# Autodesk Inventor assembly: パネル型スカラアームMISUMIアルミフレーム作成Ver
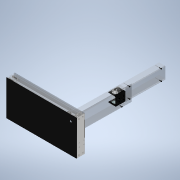
[picture p0: Inventor's stored thumbnail of the model, 180x180]
Saved by Autodesk Inventor 2022 (Build 260153000, 153)
## iProperties
Created: 2022-12-05
Part Number: パネル型スカラアームMISUMIアルミフレーム作成Ver
Document SubType Name: Assembly
Designer: tdn82
Author: tdn82
## Documents named in this file (29)
- C:\Users\tdn82\OneDrive\ドキュメント\Inventor\卒業研究パネル型スカラアーム\GrabCAD\panel-type-scalar-arm\パネル型スカラアーム\パネル型スカラアームMISUMIアルミフレーム作成Ver.iam
- C:\Users\tdn82\OneDrive\ドキュメント\Inventor\卒業研究パネル型スカラアーム\GrabCAD\panel-type-scalar-arm\パネル型スカラアーム\HFSF5-2040-180-LWH-RWH.ipt
- C:\Users\tdn82\OneDrive\ドキュメント\Inventor\卒業研究パネル型スカラアーム\GrabCAD\panel-type-scalar-arm\パネル型スカラアーム\HFSF5-2040-320-TPW.ipt
- C:\Users\tdn82\OneDrive\ドキュメント\Inventor\卒業研究パネル型スカラアーム\GrabCAD\panel-type-scalar-arm\パネル型スカラアーム\後ろカバー.ipt
- C:\Users\tdn82\OneDrive\ドキュメント\Inventor\卒業研究パネル型スカラアーム\GrabCAD\panel-type-scalar-arm\パネル型スカラアーム\サーボモータ固定用１軸目.ipt
- C:\Users\tdn82\OneDrive\ドキュメント\Inventor\卒業研究パネル型スカラアーム\GrabCAD\panel-type-scalar-arm\パネル型スカラアーム\サーボモータB3M-SC-1170-AB3M1100_scale.ipt
- C:\Users\tdn82\OneDrive\ドキュメント\Inventor\卒業研究パネル型スカラアーム\GrabCAD\panel-type-scalar-arm\パネル型スカラアーム\サーボ固定パーツ３Dプリンタ出力実験\サーボモータ固定用２軸目3mm改.ipt
- C:\Users\tdn82\OneDrive\ドキュメント\Inventor\卒業研究パネル型スカラアーム\GrabCAD\panel-type-scalar-arm\パネル型スカラアーム\横長2ndフラットバー上 アルミフレーム用.ipt
- C:\Users\tdn82\OneDrive\ドキュメント\Inventor\卒業研究パネル型スカラアーム\GrabCAD\panel-type-scalar-arm\パネル型スカラアーム\前カバー中盤左アーム固定.ipt
- C:\Users\tdn82\OneDrive\ドキュメント\Inventor\卒業研究パネル型スカラアーム\GrabCAD\panel-type-scalar-arm\パネル型スカラアーム\アルミフリーホーン02137_AluminumFreeHornWithBearing_B3M_6000.ipt
- C:\Users\tdn82\OneDrive\ドキュメント\Inventor\卒業研究パネル型スカラアーム\GrabCAD\panel-type-scalar-arm\パネル型スカラアーム\横長3rdフラットバー下.ipt
- C:\Users\tdn82\OneDrive\ドキュメント\Inventor\卒業研究パネル型スカラアーム\GrabCAD\panel-type-scalar-arm\パネル型スカラアーム\横長2ndフラットバー下 アルミフレーム用.ipt
- C:\Users\tdn82\OneDrive\ドキュメント\Inventor\卒業研究パネル型スカラアーム\GrabCAD\panel-type-scalar-arm\パネル型スカラアーム\前カバー中段右.ipt
- C:\Users\tdn82\OneDrive\ドキュメント\Inventor\卒業研究パネル型スカラアーム\GrabCAD\panel-type-scalar-arm\パネル型スカラアーム\前上カバーサーボ隠し.ipt
- C:\Users\tdn82\OneDrive\ドキュメント\Inventor\卒業研究パネル型スカラアーム\GrabCAD\panel-type-scalar-arm\パネル型スカラアーム\前下カバーサーボ隠し.ipt
- C:\Users\tdn82\OneDrive\ドキュメント\Inventor\卒業研究パネル型スカラアーム\GrabCAD\panel-type-scalar-arm\パネル型スカラアーム\ベアリング.ipt
- C:\Users\tdn82\OneDrive\ドキュメント\Inventor\卒業研究パネル型スカラアーム\GrabCAD\panel-type-scalar-arm\パネル型スカラアーム\シャフト.ipt
- C:\Users\tdn82\OneDrive\ドキュメント\Inventor\卒業研究パネル型スカラアーム\GrabCAD\panel-type-scalar-arm\パネル型スカラアーム\シャフトカラー.ipt
- C:\Users\tdn82\OneDrive\ドキュメント\Inventor\卒業研究パネル型スカラアーム\GrabCAD\panel-type-scalar-arm\パネル型スカラアーム\三段目アクリル板.ipt
- C:\Users\tdn82\OneDrive\ドキュメント\Inventor\卒業研究パネル型スカラアーム\GrabCAD\panel-type-scalar-arm\パネル型スカラアーム\シャフトカラー.iam
- C:\Users\tdn82\OneDrive\ドキュメント\Inventor\卒業研究パネル型スカラアーム\GrabCAD\panel-type-scalar-arm\パネル型スカラアーム\HFSF5-2040-180-LWH-RWH Left.ipt
- C:\Users\tdn82\OneDrive\ドキュメント\Inventor\卒業研究パネル型スカラアーム\GrabCAD\panel-type-scalar-arm\パネル型スカラアーム\HFS5-2040-180-Z5-YA10-YB170-Left.ipt
- C:\Users\tdn82\OneDrive\ドキュメント\Inventor\卒業研究パネル型スカラアーム\GrabCAD\panel-type-scalar-arm\パネル型スカラアーム\CBE5-20.ipt
- C:\Users\tdn82\OneDrive\ドキュメント\Inventor\卒業研究パネル型スカラアーム\GrabCAD\panel-type-scalar-arm\パネル型スカラアーム\CSPPN-ST-M3-6_STEP_AP203AP214\CSPPN-STC-M3-6CSPPN-ST-M3-6_203.ipt
- C:\Users\tdn82\OneDrive\ドキュメント\Inventor\卒業研究パネル型スカラアーム\GrabCAD\panel-type-scalar-arm\パネル型スカラアーム\CBE3-20.ipt
- C:\Users\tdn82\OneDrive\ドキュメント\Inventor\卒業研究パネル型スカラアーム\GrabCAD\panel-type-scalar-arm\パネル型スカラアーム\CSPSL-ST3W-M2_6-10_STEP_AP203AP214\サーボホーンとアーム固定するねじCSPSL-ST3W-M2_6-10_203.ipt
- C:\Users\tdn82\OneDrive\ドキュメント\Inventor\卒業研究パネル型スカラアーム\GrabCAD\panel-type-scalar-arm\パネル型スカラアーム\CSPPN-ST-M2_6-18_STEP_AP203AP214\CSPPN-ST-M2_6-18_203.ipt
- C:\Users\tdn82\OneDrive\ドキュメント\Inventor\卒業研究パネル型スカラアーム\GrabCAD\panel-type-scalar-arm\パネル型スカラアーム\CSPPN-ST-M3-6_STEP_AP203AP214\CSPPN-STC-M3-6CSPPN-ST-M3-10_203 - コピー.ipt
- C:\Users\tdn82\OneDrive\ドキュメント\Inventor\卒業研究パネル型スカラアーム\GrabCAD\panel-type-scalar-arm\パネル型スカラアーム\HFSF5-2040-180-LMH-RMH.ipt
## Components (69 placed, 27 different names)
1. HFSF5-2040-180-LWH-RWH:2 — 挿入:5, 挿入:7, メイト:4, フラッシュ:1, メイト:12, メイト:14, メイト:26, フラッシュ:4, 挿入:39, 挿入:40
2. HFSF5-2040-320-TPW:1 — 挿入:5, 挿入:7, メイト:1, メイト:5, メイト:13, 挿入:38, 挿入:44, 挿入:92
3. HFSF5-2040-320-TPW:2 — 挿入:39, 挿入:40, 挿入:41, 挿入:45, 挿入:46, 挿入:93
4. 後ろカバー:1 — メイト:1, メイト:26, フラッシュ:4
5. サーボモータ固定用１軸目:1 — 挿入:11, 挿入:12, 挿入:13, メイト:4, フラッシュ:1, 挿入:78, 挿入:79, 挿入:80
6. サーボモータB3M-SC-1170-AB3M1100_scale:1 — 挿入:11, 挿入:12, 挿入:13, メイト:5, 挿入:14
7. サーボモータ固定用２軸目3mm改:1 — 挿入:15, 挿入:16, 挿入:18, 挿入:19, 挿入:75, 挿入:76, 挿入:77
8. 横長2ndフラットバー上 アルミフレーム用:1 — 挿入:14, メイト:7, フラッシュ:3, メイト:19, 挿入:67, 挿入:68, 挿入:69, 挿入:70
9. 前カバー中盤左アーム固定:1 — メイト:7, 挿入:15, 挿入:16, 挿入:23, 挿入:24, フラッシュ:3, メイト:19, 挿入:72, 挿入:73, 挿入:74, 挿入:81, 挿入:82, 挿入:83, 挿入:84, 挿入:91, 角度:1
10. サーボモータB3M-SC-1170-AB3M1100_scale:2 — 挿入:17, 挿入:18, 挿入:19, メイト:22, 挿入:32
11. アルミフリーホーン02137_AluminumFreeHornWithBearing_B3M_6000:1 — 挿入:17, 挿入:30, 挿入:31
12. 横長3rdフラットバー下:1 — フラッシュ:2, メイト:22, 挿入:32, メイト:25, 挿入:59, 挿入:60, 挿入:61, 挿入:62
13. 横長3rdフラットバー下:2 — フラッシュ:2, 挿入:30, 挿入:31, メイト:23, メイト:24, 挿入:63, 挿入:64, 挿入:65, 挿入:66
14. 横長2ndフラットバー下 アルミフレーム用:1 — 挿入:23, 挿入:24, 挿入:26
15. 前カバー中段右:1 — メイト:12, メイト:15, メイト:16, メイト:17, メイト:18
16. 前上カバーサーボ隠し:1 — メイト:13, メイト:14, メイト:15, メイト:16
17. 前下カバーサーボ隠し:1 — メイト:17, メイト:18
18. ベアリング:1 — 挿入:26, 挿入:35
19. シャフト:1 — 挿入:36
20. シャフトカラー:2 — 挿入:35, 挿入:36, 挿入:37
21. 三段目アクリル板:1 — メイト:23, メイト:24, メイト:25, 挿入:85, 挿入:86, 挿入:87, 挿入:88, 角度:1
22. シャフトカラー:3 [sub-assembly] — 挿入:37, 挿入:46, 挿入:89, 挿入:90
23. HFSF5-2040-180-LWH-RWH Left:1 — 挿入:38, 挿入:41
24. HFS5-2040-180-Z5-YA10-YB170-Left:1 — 挿入:44, 挿入:45, 挿入:47, 挿入:48, 挿入:49, 挿入:50
25. CBE5-20:1 — 挿入:48
26. CBE5-20:2 — 挿入:47
27. CBE5-20:3 — 挿入:49
28. CBE5-20:4 — 挿入:50
29. CBE5-20:5 — 挿入:95
30. CBE5-20:6 — 挿入:94
31. CBE5-20:7 — 挿入:98
32. CBE5-20:8 — 挿入:97
33. CBE3-20:1 — 挿入:101
34. CBE3-20:2 — 挿入:102
35. CBE3-20:3 — 挿入:99
36. CBE3-20:4 — 挿入:100
37. サーボホーンとアーム固定するねじCSPSL-ST3W-M2_6-10_203:1 — 挿入:59
38. サーボホーンとアーム固定するねじCSPSL-ST3W-M2_6-10_203:2 — 挿入:61
39. サーボホーンとアーム固定するねじCSPSL-ST3W-M2_6-10_203:3 — 挿入:62
40. サーボホーンとアーム固定するねじCSPSL-ST3W-M2_6-10_203:4 — 挿入:60
41. サーボホーンとアーム固定するねじCSPSL-ST3W-M2_6-10_203:5 — 挿入:68
42. サーボホーンとアーム固定するねじCSPSL-ST3W-M2_6-10_203:6 — 挿入:67
43. サーボホーンとアーム固定するねじCSPSL-ST3W-M2_6-10_203:7 — 挿入:69
44. サーボホーンとアーム固定するねじCSPSL-ST3W-M2_6-10_203:8 — 挿入:70
45. サーボホーンとアーム固定するねじCSPSL-ST3W-M2_6-10_203:9 — 挿入:63
46. サーボホーンとアーム固定するねじCSPSL-ST3W-M2_6-10_203:10 — 挿入:64
47. サーボホーンとアーム固定するねじCSPSL-ST3W-M2_6-10_203:11 — 挿入:66
48. サーボホーンとアーム固定するねじCSPSL-ST3W-M2_6-10_203:12 — 挿入:65
49. CSPPN-STC-M3-6CSPPN-ST-M3-6_203:2 — 挿入:72
50. CSPPN-STC-M3-6CSPPN-ST-M3-6_203:3 — 挿入:74
51. CSPPN-STC-M3-6CSPPN-ST-M3-6_203:4 — 挿入:73
52. CSPPN-ST-M2_6-18_203:2 — 挿入:77
53. CSPPN-ST-M2_6-18_203:3 — 挿入:76
54. CSPPN-ST-M2_6-18_203:4 — 挿入:75
55. CSPPN-ST-M2_6-18_203:5 — 挿入:78
56. CSPPN-ST-M2_6-18_203:6 — 挿入:80
57. CSPPN-ST-M2_6-18_203:8 — 挿入:79
58. CSPPN-STC-M3-6CSPPN-ST-M3-10_203 - コピー:1 — 挿入:81
59. CSPPN-STC-M3-6CSPPN-ST-M3-10_203 - コピー:2 — 挿入:82
60. CSPPN-STC-M3-6CSPPN-ST-M3-10_203 - コピー:3 — 挿入:89
61. CSPPN-STC-M3-6CSPPN-ST-M3-10_203 - コピー:4 — 挿入:85
62. CSPPN-STC-M3-6CSPPN-ST-M3-10_203 - コピー:5 — 挿入:83
63. CSPPN-STC-M3-6CSPPN-ST-M3-10_203 - コピー:6 — 挿入:84
64. CSPPN-STC-M3-6CSPPN-ST-M3-10_203 - コピー:7 — 挿入:86
65. CSPPN-STC-M3-6CSPPN-ST-M3-10_203 - コピー:8 — 挿入:87
66. CSPPN-STC-M3-6CSPPN-ST-M3-10_203 - コピー:9 — 挿入:90
67. CSPPN-STC-M3-6CSPPN-ST-M3-10_203 - コピー:10 — 挿入:88
68. CSPPN-STC-M3-6CSPPN-ST-M3-6_203:5 — 挿入:91
69. HFSF5-2040-180-LMH-RMH:1 — 挿入:92, 挿入:93, 挿入:94, 挿入:95, 挿入:97, 挿入:98, 挿入:99, 挿入:100, 挿入:101, 挿入:102
## Relationships (95: Insert 73, Mate 17, Flush 4, Angle 1)
- 挿入:5 [Insert]: HFSF5-2040-180-LWH-RWH:2 ↔ HFSF5-2040-320-TPW:1
- 挿入:7 [Insert]: HFSF5-2040-180-LWH-RWH:2 ↔ HFSF5-2040-320-TPW:1
- メイト:1 [Mate]: HFSF5-2040-320-TPW:1 ↔ 後ろカバー:1
- 挿入:11 [Insert]: サーボモータ固定用１軸目:1 ↔ サーボモータB3M-SC-1170-AB3M1100_scale:1
- 挿入:12 [Insert]: サーボモータ固定用１軸目:1 ↔ サーボモータB3M-SC-1170-AB3M1100_scale:1
- 挿入:13 [Insert]: サーボモータ固定用１軸目:1 ↔ サーボモータB3M-SC-1170-AB3M1100_scale:1
- メイト:4 [Mate]: HFSF5-2040-180-LWH-RWH:2 ↔ サーボモータ固定用１軸目:1
- フラッシュ:1 [Flush]: HFSF5-2040-180-LWH-RWH:2 ↔ サーボモータ固定用１軸目:1
- メイト:5 [Mate] (0.5 mm): HFSF5-2040-320-TPW:1 ↔ サーボモータB3M-SC-1170-AB3M1100_scale:1
- 挿入:14 [Insert]: サーボモータB3M-SC-1170-AB3M1100_scale:1 ↔ 横長2ndフラットバー上 アルミフレーム用:1
- メイト:7 [Mate]: 横長2ndフラットバー上 アルミフレーム用:1 ↔ 前カバー中盤左アーム固定:1
- 挿入:15 [Insert]: サーボモータ固定用２軸目3mm改:1 ↔ 前カバー中盤左アーム固定:1
- 挿入:16 [Insert]: サーボモータ固定用２軸目3mm改:1 ↔ 前カバー中盤左アーム固定:1
- 挿入:17 [Insert]: サーボモータB3M-SC-1170-AB3M1100_scale:2 ↔ アルミフリーホーン02137_AluminumFreeHornWithBearing_B3M_6000:1
- 挿入:18 [Insert]: サーボモータ固定用２軸目3mm改:1 ↔ サーボモータB3M-SC-1170-AB3M1100_scale:2
- 挿入:19 [Insert]: サーボモータ固定用２軸目3mm改:1 ↔ サーボモータB3M-SC-1170-AB3M1100_scale:2
- フラッシュ:2 [Flush]: 横長3rdフラットバー下:1 ↔ 横長3rdフラットバー下:2
- 挿入:23 [Insert]: 前カバー中盤左アーム固定:1 ↔ 横長2ndフラットバー下 アルミフレーム用:1
- 挿入:24 [Insert]: 前カバー中盤左アーム固定:1 ↔ 横長2ndフラットバー下 アルミフレーム用:1
- メイト:12 [Mate]: HFSF5-2040-180-LWH-RWH:2 ↔ 前カバー中段右:1
- メイト:13 [Mate] (-1 mm): HFSF5-2040-320-TPW:1 ↔ 前上カバーサーボ隠し:1
- メイト:14 [Mate] (-1 mm): HFSF5-2040-180-LWH-RWH:2 ↔ 前上カバーサーボ隠し:1
- メイト:15 [Mate]: 前カバー中段右:1 ↔ 前上カバーサーボ隠し:1
- メイト:16 [Mate]: 前カバー中段右:1 ↔ 前上カバーサーボ隠し:1
- メイト:17 [Mate]: 前カバー中段右:1 ↔ 前下カバーサーボ隠し:1
- メイト:18 [Mate]: 前カバー中段右:1 ↔ 前下カバーサーボ隠し:1
- フラッシュ:3 [Flush] (29 mm): 横長2ndフラットバー上 アルミフレーム用:1 ↔ 前カバー中盤左アーム固定:1
- メイト:19 [Mate]: 横長2ndフラットバー上 アルミフレーム用:1 ↔ 前カバー中盤左アーム固定:1
- 挿入:26 [Insert]: 横長2ndフラットバー下 アルミフレーム用:1 ↔ ベアリング:1
- メイト:22 [Mate]: サーボモータB3M-SC-1170-AB3M1100_scale:2 ↔ 横長3rdフラットバー下:1
- 挿入:30 [Insert]: アルミフリーホーン02137_AluminumFreeHornWithBearing_B3M_6000:1 ↔ 横長3rdフラットバー下:2
- 挿入:31 [Insert]: アルミフリーホーン02137_AluminumFreeHornWithBearing_B3M_6000:1 ↔ 横長3rdフラットバー下:2
- 挿入:32 [Insert]: サーボモータB3M-SC-1170-AB3M1100_scale:2 ↔ 横長3rdフラットバー下:1
- メイト:23 [Mate]: 横長3rdフラットバー下:2 ↔ 三段目アクリル板:1
- メイト:24 [Mate]: 横長3rdフラットバー下:2 ↔ 三段目アクリル板:1
- メイト:25 [Mate]: 横長3rdフラットバー下:1 ↔ 三段目アクリル板:1
- メイト:26 [Mate]: HFSF5-2040-180-LWH-RWH:2 ↔ 後ろカバー:1
- フラッシュ:4 [Flush]: HFSF5-2040-180-LWH-RWH:2 ↔ 後ろカバー:1
- 挿入:35 [Insert]: ベアリング:1 ↔ シャフトカラー:2
- 挿入:36 [Insert] (-5 mm): シャフト:1 ↔ シャフトカラー:2
- 挿入:37 [Insert] (2 mm): シャフトカラー:2 ↔ シャフトカラー:3
- 挿入:38 [Insert]: HFSF5-2040-320-TPW:1 ↔ HFSF5-2040-180-LWH-RWH Left:1
- 挿入:39 [Insert]: HFSF5-2040-180-LWH-RWH:2 ↔ HFSF5-2040-320-TPW:2
- 挿入:40 [Insert]: HFSF5-2040-180-LWH-RWH:2 ↔ HFSF5-2040-320-TPW:2
- 挿入:41 [Insert]: HFSF5-2040-320-TPW:2 ↔ HFSF5-2040-180-LWH-RWH Left:1
- 挿入:44 [Insert] (6 mm): HFSF5-2040-320-TPW:1 ↔ HFS5-2040-180-Z5-YA10-YB170-Left:1
- 挿入:45 [Insert] (6 mm): HFSF5-2040-320-TPW:2 ↔ HFS5-2040-180-Z5-YA10-YB170-Left:1
- 挿入:46 [Insert]: HFSF5-2040-320-TPW:2 ↔ シャフトカラー:3
- 挿入:47 [Insert]: HFS5-2040-180-Z5-YA10-YB170-Left:1 ↔ CBE5-20:2
- 挿入:48 [Insert]: HFS5-2040-180-Z5-YA10-YB170-Left:1 ↔ CBE5-20:1
- 挿入:49 [Insert]: HFS5-2040-180-Z5-YA10-YB170-Left:1 ↔ CBE5-20:3
- 挿入:50 [Insert]: HFS5-2040-180-Z5-YA10-YB170-Left:1 ↔ CBE5-20:4
- 挿入:59 [Insert]: 横長3rdフラットバー下:1 ↔ サーボホーンとアーム固定するねじCSPSL-ST3W-M2_6-10_203:1
- 挿入:60 [Insert]: 横長3rdフラットバー下:1 ↔ サーボホーンとアーム固定するねじCSPSL-ST3W-M2_6-10_203:4
- 挿入:61 [Insert]: 横長3rdフラットバー下:1 ↔ サーボホーンとアーム固定するねじCSPSL-ST3W-M2_6-10_203:2
- 挿入:62 [Insert]: 横長3rdフラットバー下:1 ↔ サーボホーンとアーム固定するねじCSPSL-ST3W-M2_6-10_203:3
- 挿入:63 [Insert]: 横長3rdフラットバー下:2 ↔ サーボホーンとアーム固定するねじCSPSL-ST3W-M2_6-10_203:9
- 挿入:64 [Insert]: 横長3rdフラットバー下:2 ↔ サーボホーンとアーム固定するねじCSPSL-ST3W-M2_6-10_203:10
- 挿入:65 [Insert]: 横長3rdフラットバー下:2 ↔ サーボホーンとアーム固定するねじCSPSL-ST3W-M2_6-10_203:12
- 挿入:66 [Insert]: 横長3rdフラットバー下:2 ↔ サーボホーンとアーム固定するねじCSPSL-ST3W-M2_6-10_203:11
- 挿入:67 [Insert]: 横長2ndフラットバー上 アルミフレーム用:1 ↔ サーボホーンとアーム固定するねじCSPSL-ST3W-M2_6-10_203:6
- 挿入:68 [Insert]: 横長2ndフラットバー上 アルミフレーム用:1 ↔ サーボホーンとアーム固定するねじCSPSL-ST3W-M2_6-10_203:5
- 挿入:69 [Insert]: 横長2ndフラットバー上 アルミフレーム用:1 ↔ サーボホーンとアーム固定するねじCSPSL-ST3W-M2_6-10_203:7
- 挿入:70 [Insert]: 横長2ndフラットバー上 アルミフレーム用:1 ↔ サーボホーンとアーム固定するねじCSPSL-ST3W-M2_6-10_203:8
- 挿入:72 [Insert]: 前カバー中盤左アーム固定:1 ↔ CSPPN-STC-M3-6CSPPN-ST-M3-6_203:2
- 挿入:73 [Insert]: 前カバー中盤左アーム固定:1 ↔ CSPPN-STC-M3-6CSPPN-ST-M3-6_203:4
- 挿入:74 [Insert]: 前カバー中盤左アーム固定:1 ↔ CSPPN-STC-M3-6CSPPN-ST-M3-6_203:3
- 挿入:75 [Insert]: サーボモータ固定用２軸目3mm改:1 ↔ CSPPN-ST-M2_6-18_203:4
- 挿入:76 [Insert]: サーボモータ固定用２軸目3mm改:1 ↔ CSPPN-ST-M2_6-18_203:3
- 挿入:77 [Insert]: サーボモータ固定用２軸目3mm改:1 ↔ CSPPN-ST-M2_6-18_203:2
- 挿入:78 [Insert]: サーボモータ固定用１軸目:1 ↔ CSPPN-ST-M2_6-18_203:5
- 挿入:79 [Insert]: サーボモータ固定用１軸目:1 ↔ CSPPN-ST-M2_6-18_203:8
- 挿入:80 [Insert]: サーボモータ固定用１軸目:1 ↔ CSPPN-ST-M2_6-18_203:6
- 挿入:81 [Insert]: 前カバー中盤左アーム固定:1 ↔ CSPPN-STC-M3-6CSPPN-ST-M3-10_203 - コピー:1
- 挿入:82 [Insert]: 前カバー中盤左アーム固定:1 ↔ CSPPN-STC-M3-6CSPPN-ST-M3-10_203 - コピー:2
- 挿入:83 [Insert]: 前カバー中盤左アーム固定:1 ↔ CSPPN-STC-M3-6CSPPN-ST-M3-10_203 - コピー:5
- 挿入:84 [Insert]: 前カバー中盤左アーム固定:1 ↔ CSPPN-STC-M3-6CSPPN-ST-M3-10_203 - コピー:6
- 挿入:85 [Insert]: 三段目アクリル板:1 ↔ CSPPN-STC-M3-6CSPPN-ST-M3-10_203 - コピー:4
- 挿入:86 [Insert]: 三段目アクリル板:1 ↔ CSPPN-STC-M3-6CSPPN-ST-M3-10_203 - コピー:7
- 挿入:87 [Insert]: 三段目アクリル板:1 ↔ CSPPN-STC-M3-6CSPPN-ST-M3-10_203 - コピー:8
- 挿入:88 [Insert]: 三段目アクリル板:1 ↔ CSPPN-STC-M3-6CSPPN-ST-M3-10_203 - コピー:10
- 挿入:89 [Insert]: シャフトカラー:3 ↔ CSPPN-STC-M3-6CSPPN-ST-M3-10_203 - コピー:3
- 挿入:90 [Insert]: シャフトカラー:3 ↔ CSPPN-STC-M3-6CSPPN-ST-M3-10_203 - コピー:9
- 挿入:91 [Insert]: 前カバー中盤左アーム固定:1 ↔ CSPPN-STC-M3-6CSPPN-ST-M3-6_203:5
- 角度:1 [Angle] (0 deg): 前カバー中盤左アーム固定:1 ↔ 三段目アクリル板:1
- 挿入:92 [Insert]: HFSF5-2040-320-TPW:1 ↔ HFSF5-2040-180-LMH-RMH:1
- 挿入:93 [Insert]: HFSF5-2040-320-TPW:2 ↔ HFSF5-2040-180-LMH-RMH:1
- 挿入:94 [Insert]: CBE5-20:6 ↔ HFSF5-2040-180-LMH-RMH:1
- 挿入:95 [Insert]: CBE5-20:5 ↔ HFSF5-2040-180-LMH-RMH:1
- 挿入:97 [Insert]: CBE5-20:8 ↔ HFSF5-2040-180-LMH-RMH:1
- 挿入:98 [Insert]: CBE5-20:7 ↔ HFSF5-2040-180-LMH-RMH:1
- 挿入:99 [Insert]: CBE3-20:3 ↔ HFSF5-2040-180-LMH-RMH:1
- 挿入:100 [Insert]: CBE3-20:4 ↔ HFSF5-2040-180-LMH-RMH:1
- 挿入:101 [Insert]: CBE3-20:1 ↔ HFSF5-2040-180-LMH-RMH:1
- 挿入:102 [Insert]: CBE3-20:2 ↔ HFSF5-2040-180-LMH-RMH:1
